# Autodesk Inventor assembly: Lath
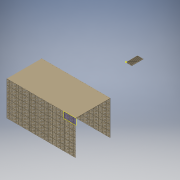
[picture p0: Inventor's stored thumbnail of the model, 180x180]
Saved by Autodesk Inventor 2018 (Build 220112000, 112)
## iProperties
Created: 2019-05-10
Part Number: Lath
Document SubType Name: Assembly
Designer: 10043883
Author: 10043883
## Documents named in this file (4)
- C:\Users\10043883\Documents\GitHub\IED-files\Lathhouse\Lath.iam
- C:\Users\10043883\Documents\GitHub\IED-files\Lathhouse\Lathhouse wall.ipt
- C:\Users\10043883\Documents\GitHub\IED-files\Lathhouse\Foor.ipt
- C:\Users\10043883\Documents\GitHub\IED-files\Lathhouse\Lathhouse roof.ipt
## Components (4 placed, 3 different names)
1. Foor:1 — Mate:1, Mate:2, Mate:3, Mate:4
2. Lathhouse wall:1 — Mate:1, Mate:2
3. Lathhouse wall:2 — Mate:3, Mate:4
4. Lathhouse roof:1
## Relationships (4: Mate 4)
- Mate:1: Foor:1 ↔ Lathhouse wall:1
- Mate:2: Foor:1 ↔ Lathhouse wall:1
- Mate:3: Foor:1 ↔ Lathhouse wall:2
- Mate:4: Foor:1 ↔ Lathhouse wall:2
